# Autodesk Inventor assembly: 車輪部分
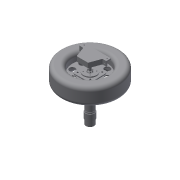
[picture p0: Inventor's stored thumbnail of the model, 180x180]
Saved by Autodesk Inventor 2020.3 (Build 243373000, 373)
## iProperties
Part Number: 車輪部分
Material: 一般
Document SubType Name: Assembly
Designer: highs
Author: highs
## Documents named in this file (17)
- C:\Users\toshi\Desktop\中の島ex\車輪部分.iam
- C:\Users\toshi\Desktop\中の島ex\車軸.ipt
- C:\Users\toshi\Desktop\中の島ex\車輪.ipt
- C:\Users\toshi\Desktop\中の島ex\車輪ハブ1.ipt
- C:\Users\toshi\Desktop\中の島ex\車軸受け板.ipt
- C:\Users\toshi\Desktop\中の島ex\ベアリング12x18.ipt
- C:\Users\toshi\Desktop\中の島ex\車軸受け板2.ipt
- C:\Users\toshi\Desktop\中の島ex\モータースペーサ.ipt
- C:\Users\toshi\Desktop\中の島ex\カップリング.ipt
- C:\Users\toshi\Desktop\中の島ex\IG42C-144.ipt
- C:\Users\toshi\Desktop\中の島ex\RS-775.ipt
- C:\Users\toshi\Desktop\中の島ex\AMT102-1.ipt
- C:\Users\toshi\Desktop\中の島ex\セットカラー.ipt
- C:\Users\toshi\Desktop\中の島ex\モータースペーサ2.ipt
- C:\Users\toshi\Desktop\中の島ex\エンコーダガード2.ipt
- C:\Users\toshi\Desktop\中の島ex\車軸受け板3.ipt
- C:\Users\toshi\Desktop\中の島ex\メカロック.ipt
## Components (20 placed, 16 different names)
1. 車軸:1 — メイト:39, メイト:46, メイト:52, メイト:53, フラッシュ:4, メイト:79, メイト:83, メイト:99, メイト:100
2. 車輪:1 — メイト:37, メイト:76, メイト:100
3. 車輪ハブ1:1 — メイト:37, メイト:76, メイト:91, メイト:92, メイト:93, メイト:94, メイト:95, メイト:97
4. 車軸受け板:1 — メイト:39, メイト:41, メイト:43, フラッシュ:2, メイト:59, メイト:82, メイト:84, フラッシュ:7, フラッシュ:8, メイト:90
5. ベアリング12x18:1 — メイト:46, メイト:57, メイト:58, メイト:78
6. ベアリング12x18:2 — メイト:41, メイト:43, メイト:77
7. カップリング:1 — メイト:52, メイト:53, メイト:56, メイト:80
8. IG42C-144:1 — メイト:54, メイト:55, メイト:56, メイト:60, メイト:61, メイト:62
9. RS-775:1 — メイト:54, メイト:55
10. 車軸受け板:2 — メイト:57, メイト:58, フラッシュ:2, メイト:59, フラッシュ:3, メイト:66, フラッシュ:4, メイト:101
11. 車軸受け板2:1 — メイト:60, メイト:61, メイト:62, フラッシュ:3, メイト:63, メイト:64, メイト:65, メイト:89
12. モータースペーサ:1 — メイト:63, メイト:64, メイト:65, メイト:66, フラッシュ:5, フラッシュ:6
13. セットカラー:1 — メイト:77, メイト:79
14. セットカラー:2 — メイト:78, メイト:80
15. AMT102-1:2 — メイト:82, メイト:83, メイト:84
16. モータースペーサ2:1 — フラッシュ:5, メイト:89, フラッシュ:6
17. エンコーダガード2:1 — フラッシュ:7, フラッシュ:8, メイト:90
18. 車軸受け板3:1 — メイト:91, メイト:92, メイト:93, メイト:96, メイト:101
19. 車軸受け板3:2 — メイト:94, メイト:95, メイト:96, メイト:98
20. メカロック:1 — メイト:97, メイト:98, メイト:99
## Relationships (48: Mate 41, Flush 7)
- メイト:37 [Mate]: 車輪:1 ↔ 車輪ハブ1:1
- メイト:39 [Mate]: 車軸:1 ↔ 車軸受け板:1
- メイト:41 [Mate]: 車軸受け板:1 ↔ ベアリング12x18:2
- メイト:43 [Mate]: 車軸受け板:1 ↔ ベアリング12x18:2
- メイト:46 [Mate]: 車軸:1 ↔ ベアリング12x18:1
- メイト:52 [Mate]: 車軸:1 ↔ カップリング:1
- メイト:53 [Mate] (-10 mm): 車軸:1 ↔ カップリング:1
- メイト:54 [Mate]: IG42C-144:1 ↔ RS-775:1
- メイト:55 [Mate]: IG42C-144:1 ↔ RS-775:1
- メイト:56 [Mate]: カップリング:1 ↔ IG42C-144:1
- メイト:57 [Mate]: ベアリング12x18:1 ↔ 車軸受け板:2
- メイト:58 [Mate]: ベアリング12x18:1 ↔ 車軸受け板:2
- フラッシュ:2 [Flush]: 車軸受け板:1 ↔ 車軸受け板:2
- メイト:59 [Mate] (108 mm): 車軸受け板:1 ↔ 車軸受け板:2
- メイト:60 [Mate]: IG42C-144:1 ↔ 車軸受け板2:1
- メイト:61 [Mate]: IG42C-144:1 ↔ 車軸受け板2:1
- メイト:62 [Mate]: IG42C-144:1 ↔ 車軸受け板2:1
- フラッシュ:3 [Flush]: 車軸受け板:2 ↔ 車軸受け板2:1
- メイト:63 [Mate]: 車軸受け板2:1 ↔ モータースペーサ:1
- メイト:64 [Mate]: 車軸受け板2:1 ↔ モータースペーサ:1
- メイト:65 [Mate] (8 mm): 車軸受け板2:1 ↔ モータースペーサ:1
- メイト:66 [Mate] (20 mm): 車軸受け板:2 ↔ モータースペーサ:1
- フラッシュ:4 [Flush] (-22 mm): 車軸:1 ↔ 車軸受け板:2
- メイト:76 [Mate]: 車輪:1 ↔ 車輪ハブ1:1
- メイト:77 [Mate]: ベアリング12x18:2 ↔ セットカラー:1
- メイト:78 [Mate]: ベアリング12x18:1 ↔ セットカラー:2
- メイト:79 [Mate]: 車軸:1 ↔ セットカラー:1
- メイト:80 [Mate]: カップリング:1 ↔ セットカラー:2
- メイト:82 [Mate]: 車軸受け板:1 ↔ AMT102-1:2
- メイト:83 [Mate]: 車軸:1 ↔ AMT102-1:2
- メイト:84 [Mate]: 車軸受け板:1 ↔ AMT102-1:2
- フラッシュ:5 [Flush]: モータースペーサ:1 ↔ モータースペーサ2:1
- メイト:89 [Mate]: 車軸受け板2:1 ↔ モータースペーサ2:1
- フラッシュ:6 [Flush]: モータースペーサ:1 ↔ モータースペーサ2:1
- フラッシュ:7 [Flush]: 車軸受け板:1 ↔ エンコーダガード2:1
- フラッシュ:8 [Flush] (30 mm): 車軸受け板:1 ↔ エンコーダガード2:1
- メイト:90 [Mate] (20 mm): 車軸受け板:1 ↔ エンコーダガード2:1
- メイト:91 [Mate]: 車輪ハブ1:1 ↔ 車軸受け板3:1
- メイト:92 [Mate]: 車輪ハブ1:1 ↔ 車軸受け板3:1
- メイト:93 [Mate]: 車輪ハブ1:1 ↔ 車軸受け板3:1
- メイト:94 [Mate]: 車輪ハブ1:1 ↔ 車軸受け板3:2
- メイト:95 [Mate]: 車輪ハブ1:1 ↔ 車軸受け板3:2
- メイト:96 [Mate]: 車軸受け板3:1 ↔ 車軸受け板3:2
- メイト:97 [Mate]: 車輪ハブ1:1 ↔ メカロック:1
- メイト:98 [Mate]: 車軸受け板3:2 ↔ メカロック:1
- メイト:99 [Mate]: 車軸:1 ↔ メカロック:1
- メイト:100 [Mate]: 車軸:1 ↔ 車輪:1
- メイト:101 [Mate] (50 mm): 車軸受け板:2 ↔ 車軸受け板3:1
